# Autodesk Inventor assembly: Assembly ReDes
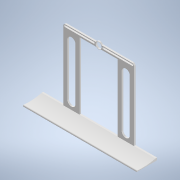
[picture p0: Inventor's stored thumbnail of the model, 180x180]
Saved by Autodesk Inventor 2020.2 (Build 242310000, 310)
## iProperties
Created: 2020-05-07
Part Number: Assembly ReDes
Document SubType Name: Assembly
Designer: Amaan Khalid
Author: Amaan Khalid
## Documents named in this file (3)
- C:\Users\Amaan Khalid\Desktop\My projects\Benq Pen Holder\Re-Deisign\Assembly ReDes.iam
- C:\Users\Amaan Khalid\Desktop\My projects\Benq Pen Holder\Re-Deisign\Pen Holder ReDes.ipt
- C:\Users\Amaan Khalid\Desktop\My projects\Benq Pen Holder\Re-Deisign\Monitor Part ReDes.ipt
## Components (2 placed, 2 different names)
1. Pen Holder ReDes:1 — Mate:1, Mate:2, Mate:3
2. Monitor Part ReDes:1 — Mate:1, Mate:2, Mate:3
## Relationships (3: Mate 3)
- Mate:1: Pen Holder ReDes:1 ↔ Monitor Part ReDes:1
- Mate:2: Pen Holder ReDes:1 ↔ Monitor Part ReDes:1
- Mate:3: Pen Holder ReDes:1 ↔ Monitor Part ReDes:1
